# Autodesk Inventor assembly: assembly_smartcare
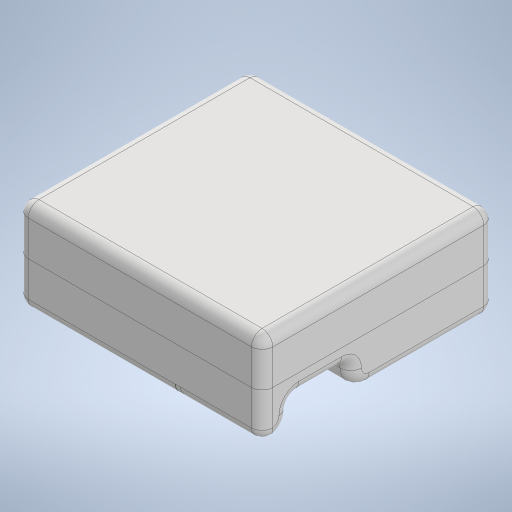
[picture p0: Inventor's stored thumbnail of the model, 512x512]
Saved by Autodesk Inventor 2023.6 (Build 276521000, 521)
## iProperties
Created: 2026-05-31
Part Number: assembly_smartcare
Document SubType Name: Assembly
Designer: Nanda
Author: Nanda
## Documents named in this file (3)
- C:\Users\Nanda\Documents\desai smart care\assembly_smartcare.iam
- C:\Users\Nanda\Documents\desai smart care\backdoor.ipt
- C:\Users\Nanda\Documents\desai smart care\Front.ipt
## Components (2 placed, 2 different names)
1. backdoor:1 — Rigid:1
2. Front:1 — Rigid:1
## Relationships (1: WeldJoint 1)
- Rigid:1 [WeldJoint]: backdoor:1 ↔ Front:1
